# Autodesk Inventor assembly: engine
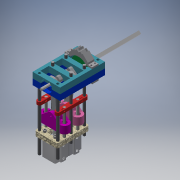
[picture p0: Inventor's stored thumbnail of the model, 180x180]
Saved by Autodesk Inventor 2017 SP1 (Build 210196100, 196)
## iProperties
Created: 2017-06-14
Part Number: engine
Document SubType Name: Assembly
Designer: RMcComber
Author: RMcComber
## Documents named in this file (22)
- C:\Users\rmccomber\Documents\st motor\two cylinder solenoid valve\engine.iam
- C:\Users\rmccomber\Documents\st motor\two cylinder solenoid valve\steam cylinder 1.iam
- C:\Users\rmccomber\Documents\st motor\two cylinder solenoid valve\con rod.ipt
- C:\Users\rmccomber\Documents\st motor\two cylinder solenoid valve\engine\Design Accelerator\Bearing1.iam
- C:\Users\rmccomber\Documents\st motor\two cylinder solenoid valve\engine\Design Accelerator\Bearing2.iam
- C:\Users\rmccomber\Documents\st motor\two cylinder solenoid valve\crank web.ipt
- C:\Users\rmccomber\Documents\st motor\two cylinder solenoid valve\frame 1.ipt
- C:\Users\rmccomber\Documents\st motor\two cylinder solenoid valve\sensor wheel.ipt
- C:\Users\rmccomber\Documents\st motor\two cylinder solenoid valve\sensor bracket coupler.ipt
- C:\Users\rmccomber\Documents\st motor\two cylinder solenoid valve\engine\Design Accelerator\Shaft1.iam
- C:\Users\rmccomber\Documents\st motor\two cylinder solenoid valve\engine\Design Accelerator\Shaft2.iam
- C:\Users\rmccomber\Documents\st motor\two cylinder solenoid valve\engine\Design Accelerator\Shaft3.iam
- C:\Users\rmccomber\Documents\st motor\two cylinder solenoid valve\engine\Design Accelerator\Shaft4.iam
- C:\Users\rmccomber\Documents\st motor\two cylinder solenoid valve\engine\Design Accelerator\Shaft5.iam
- C:\Users\rmccomber\Documents\st motor\two cylinder solenoid valve\frame rod 1.ipt
- C:\Users\rmccomber\Documents\st motor\two cylinder solenoid valve\engine\Design Accelerator\Bolted Connection5.iam
- C:\Users\rmccomber\Documents\st motor\two cylinder solenoid valve\crank web2.ipt
- C:\Users\rmccomber\Documents\st motor\two cylinder solenoid valve\hall follower.ipt
- C:\Users\rmccomber\Documents\st motor\two cylinder shaft drive 2\cylinder frame.ipt
- C:\Users\rmccomber\Documents\st motor\two cylinder shaft drive 2\combo cross head.ipt
- C:\Users\rmccomber\Documents\st motor\two cylinder shaft drive 2\guide rod.ipt
- C:\Users\rmccomber\Documents\st motor\two cylinder shaft drive 2\guide rod mount.ipt
## Components (47 placed, 16 different names)
1. steam cylinder 1:1 [sub-assembly] — Mate:1, Flush:1, Flush:2, Mate:32, Mate:238, Mate:239
2. steam cylinder 1:2 [sub-assembly] — Mate:1, Flush:1, Flush:2, Mate:27, Mate:30, Mate:31, Mate:242, Mate:243
3. combo cross head:2 — Mate:242, Mate:243, Mate:244, Mate:245
4. combo cross head:1 — Mate:238, Mate:239, Mate:240, Mate:241
5. con rod:1 — Flush:4, Mate:13, Mate:16, Mate:18, Flush:55, Mate:245
6. con rod:2 — Mate:12, Mate:21, Mate:23, Mate:40, Flush:46, Flush:48, Mate:109, Mate:241
7. Bearing:2 [sub-assembly] — Mate:22, Mate:24, Mate:40, Flush:48, Mate:109
8. Bearing:1 [sub-assembly] — Flush:4, Mate:13, Mate:17, Mate:19
9. Bearing:1 [sub-assembly] — Mate:12, Flush:46
10. crank web:1 — Mate:16, Mate:17, Angle:3, Mate:67, Angle:13, Mate:223, Angle:15, Mate:224
11. crank web2:1 — Mate:18, Mate:19, Mate:86, Mate:87, Angle:15, Mate:225
12. crank web:3 — Mate:23, Mate:24, Angle:3, Mate:66, Mate:90, Mate:91, Angle:13, Flush:62, Mate:220, Mate:221, Angle:16
13. crank web:4 — Mate:21, Mate:22, Mate:219, Angle:14, Angle:16, Mate:227, Mate:228
14. frame 1:1 — Mate:27, Mate:33, Mate:34, Mate:63, Mate:66, Mate:67, Mate:229, Flush:63, Flush:64, Mate:231, Mate:234, Flush:65, Mate:235, Flush:68, Mate:247
15. cylinder frame:1 — Mate:30, Mate:31, Mate:32, Mate:33, Mate:34, Mate:138, Mate:139, Mate:140, Mate:141, Mate:142, Mate:143, Mate:144, Mate:145, Mate:146, Mate:147, Mate:148, Mate:149, Mate:150, Mate:151, Mate:152, Mate:153, Mate:240, Mate:244, Flush:73, Mate:249, Flush:74, Mate:250, Flush:76, Mate:253, Flush:77, Mate:254
16. frame 1:2 — Mate:63, Flush:58, Mate:154, Flush:59, Flush:60, Mate:155, Mate:156, Flush:61, Mate:157, Flush:63, Mate:230, Flush:64, Mate:236, Mate:237, Flush:70, Flush:71
17. sensor wheel:1 — Mate:231, Mate:232, Flush:66, Mate:255, Mate:257, Angle:17
18. sensor bracket coupler:1 — Mate:256, Mate:257, Angle:17
19. Shaft:1 [sub-assembly] — Flush:55, Mate:225, Mate:230
20. Shaft:2 [sub-assembly] — Mate:86, Mate:87
21. Shaft:3 [sub-assembly] — Flush:62, Mate:220, Mate:221, Mate:223, Mate:224
22. Shaft:4 [sub-assembly] — Mate:90, Mate:91
23. Shaft:5 [sub-assembly] — Mate:219, Angle:14, Mate:227, Mate:228, Mate:232, Mate:255, Mate:256
24. frame rod 1:1 — Flush:60, Mate:156, Mate:251
25. frame rod 1:2 — Flush:59, Mate:155
26. frame rod 1:3 — Flush:58, Mate:154, Mate:246
27. frame rod 1:4 — Flush:61, Mate:157
28. frame rod 1:5 — Mate:229, Mate:252
29. frame rod 1:6 — Mate:247, Mate:248
30. Bolted Connection:13 [sub-assembly] — Mate:138, Mate:139
31. Bolted Connection:14 [sub-assembly] — Mate:146, Mate:147
32. Bolted Connection:15 [sub-assembly] — Mate:148, Mate:149
33. Bolted Connection:16 [sub-assembly] — Mate:142, Mate:143
34. Bolted Connection:17 [sub-assembly] — Mate:140, Mate:141
35. Bolted Connection:18 [sub-assembly] — Mate:144, Mate:145
36. Bolted Connection:19 [sub-assembly] — Mate:152, Mate:153
37. Bolted Connection:20 [sub-assembly] — Mate:150, Mate:151
38. hall follower:1 — Mate:234, Flush:65, Flush:66, Flush:67, Flush:72
39. hall follower:2 — Mate:235, Flush:67, Flush:68
40. hall follower:3 — Mate:236, Flush:69, Flush:71, Flush:72
41. hall follower:4 — Mate:237, Flush:69, Flush:70
42. guide rod:1 — Mate:253, Flush:77, Flush:78
43. guide rod:2 — Flush:73, Mate:254
44. guide rod:3 — Mate:250, Flush:76
45. guide rod:4 — Mate:249, Flush:74, Flush:75
46. guide rod mount:1 — Mate:246, Mate:248, Flush:75
47. guide rod mount:2 — Mate:251, Mate:252, Flush:78
## Relationships (115: Mate 82, Flush 27, Angle 6)
- Mate:1: steam cylinder 1:1 ↔ steam cylinder 1:2
- Flush:1: steam cylinder 1:1 ↔ steam cylinder 1:2
- Flush:2: steam cylinder 1:1 ↔ steam cylinder 1:2
- Mate:12: con rod:2 ↔ Bearing:1
- Flush:4: con rod:1 ↔ Bearing:1
- Mate:13: con rod:1 ↔ Bearing:1
- Mate:16: con rod:1 ↔ crank web:1
- Mate:17: Bearing:1 ↔ crank web:1
- Mate:18: con rod:1 ↔ crank web2:1
- Mate:19: Bearing:1 ↔ crank web2:1
- Mate:21: con rod:2 ↔ crank web:4
- Mate:22: Bearing:2 ↔ crank web:4
- Mate:23: con rod:2 ↔ crank web:3
- Mate:24: Bearing:2 ↔ crank web:3
- Angle:3 (-90 deg): crank web:1 ↔ crank web:3
- Mate:27 (139 mm): steam cylinder 1:2 ↔ frame 1:1
- Mate:30: steam cylinder 1:2 ↔ cylinder frame:1
- Mate:31: steam cylinder 1:2 ↔ cylinder frame:1
- Mate:32: steam cylinder 1:1 ↔ cylinder frame:1
- Mate:33: frame 1:1 ↔ cylinder frame:1
- Mate:34: frame 1:1 ↔ cylinder frame:1
- Mate:40: con rod:2 ↔ Bearing:2
- Flush:46: con rod:2 ↔ Bearing:1
- Flush:48: con rod:2 ↔ Bearing:2
- Mate:63: frame 1:1 ↔ frame 1:2
- Mate:66: crank web:3 ↔ frame 1:1
- Mate:67: crank web:1 ↔ frame 1:1
- Flush:55: con rod:1 ↔ Shaft:1
- Mate:86: crank web2:1 ↔ Shaft:2
- Mate:87: crank web2:1 ↔ Shaft:2
- Mate:90: crank web:3 ↔ Shaft:4
- Mate:91: crank web:3 ↔ Shaft:4
- Angle:13 (0 deg): crank web:1 ↔ crank web:3
- Mate:109: con rod:2 ↔ Bearing:2
- Mate:138: cylinder frame:1 ↔ Bolted Connection:13
- Mate:139: cylinder frame:1 ↔ Bolted Connection:13
- Mate:140: cylinder frame:1 ↔ Bolted Connection:17
- Mate:141: cylinder frame:1 ↔ Bolted Connection:17
- Mate:142: cylinder frame:1 ↔ Bolted Connection:16
- Mate:143: cylinder frame:1 ↔ Bolted Connection:16
- Mate:144: cylinder frame:1 ↔ Bolted Connection:18
- Mate:145: cylinder frame:1 ↔ Bolted Connection:18
- Mate:146: cylinder frame:1 ↔ Bolted Connection:14
- Mate:147: cylinder frame:1 ↔ Bolted Connection:14
- Mate:148: cylinder frame:1 ↔ Bolted Connection:15
- Mate:149: cylinder frame:1 ↔ Bolted Connection:15
- Mate:150: cylinder frame:1 ↔ Bolted Connection:20
- Mate:151: cylinder frame:1 ↔ Bolted Connection:20
- Mate:152: cylinder frame:1 ↔ Bolted Connection:19
- Mate:153: cylinder frame:1 ↔ Bolted Connection:19
- Flush:58 (-10 mm): frame 1:2 ↔ frame rod 1:3
- Mate:154: frame 1:2 ↔ frame rod 1:3
- Flush:59 (-10 mm): frame 1:2 ↔ frame rod 1:2
- Flush:60 (-10 mm): frame 1:2 ↔ frame rod 1:1
- Mate:155: frame 1:2 ↔ frame rod 1:2
- Mate:156: frame 1:2 ↔ frame rod 1:1
- Flush:61 (-10 mm): frame 1:2 ↔ frame rod 1:4
- Mate:157: frame 1:2 ↔ frame rod 1:4
- Mate:219: crank web:4 ↔ Shaft:5
- Angle:14 (0 deg): crank web:4 ↔ Shaft:5
- Flush:62: crank web:3 ↔ Shaft:3
- Mate:220: crank web:3 ↔ Shaft:3
- Mate:221: crank web:3 ↔ Shaft:3
- Mate:223: crank web:1 ↔ Shaft:3
- Angle:15 (0 deg): crank web:1 ↔ crank web2:1
- Mate:224: crank web:1 ↔ Shaft:3
- Angle:16 (0 deg): crank web:3 ↔ crank web:4
- Mate:225: crank web2:1 ↔ Shaft:1
- Mate:227: crank web:4 ↔ Shaft:5
- Mate:228: crank web:4 ↔ Shaft:5
- Mate:229: frame 1:1 ↔ frame rod 1:5
- Flush:63: frame 1:1 ↔ frame 1:2
- Mate:230: frame 1:2 ↔ Shaft:1
- Flush:64: frame 1:1 ↔ frame 1:2
- Mate:231 (10 mm): frame 1:1 ↔ sensor wheel:1
- Mate:232: sensor wheel:1 ↔ Shaft:5
- Mate:234: frame 1:1 ↔ hall follower:1
- Flush:65: frame 1:1 ↔ hall follower:1
- Flush:66 (-6 mm): sensor wheel:1 ↔ hall follower:1
- Mate:235: frame 1:1 ↔ hall follower:2
- Flush:67: hall follower:1 ↔ hall follower:2
- Flush:68: frame 1:1 ↔ hall follower:2
- Mate:236: frame 1:2 ↔ hall follower:3
- Mate:237: frame 1:2 ↔ hall follower:4
- Flush:69: hall follower:3 ↔ hall follower:4
- Flush:70: frame 1:2 ↔ hall follower:4
- Flush:71: frame 1:2 ↔ hall follower:3
- Flush:72: hall follower:1 ↔ hall follower:3
- Mate:238 (15 mm): steam cylinder 1:1 ↔ combo cross head:1
- Mate:239: steam cylinder 1:1 ↔ combo cross head:1
- Mate:240: combo cross head:1 ↔ cylinder frame:1
- Mate:241: combo cross head:1 ↔ con rod:2
- Mate:242 (10 mm): steam cylinder 1:2 ↔ combo cross head:2
- Mate:243: steam cylinder 1:2 ↔ combo cross head:2
- Mate:244: combo cross head:2 ↔ cylinder frame:1
- Mate:245: combo cross head:2 ↔ con rod:1
- Mate:246: frame rod 1:3 ↔ guide rod mount:1
- Mate:247: frame 1:1 ↔ frame rod 1:6
- Mate:248: frame rod 1:6 ↔ guide rod mount:1
- Flush:73: cylinder frame:1 ↔ guide rod:2
- Mate:249: cylinder frame:1 ↔ guide rod:4
- Flush:74: cylinder frame:1 ↔ guide rod:4
- Flush:75: guide rod:4 ↔ guide rod mount:1
- Mate:250: cylinder frame:1 ↔ guide rod:3
- Flush:76: cylinder frame:1 ↔ guide rod:3
- Mate:251: frame rod 1:1 ↔ guide rod mount:2
- Mate:252: frame rod 1:5 ↔ guide rod mount:2
- Mate:253: cylinder frame:1 ↔ guide rod:1
- Flush:77: cylinder frame:1 ↔ guide rod:1
- Flush:78: guide rod:1 ↔ guide rod mount:2
- Mate:254: cylinder frame:1 ↔ guide rod:2
- Mate:255: sensor wheel:1 ↔ Shaft:5
- Mate:256: sensor bracket coupler:1 ↔ Shaft:5
- Mate:257: sensor wheel:1 ↔ sensor bracket coupler:1
- Angle:17 (0 deg): sensor wheel:1 ↔ sensor bracket coupler:1
